# Autodesk Inventor assembly: Assembly1
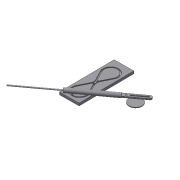
[picture p0: Inventor's stored thumbnail of the model, 180x180]
Saved by Autodesk Inventor 2017 (Build 210142000, 142)
## iProperties
Created: 2019-07-04
Part Number: Assembly1
Document SubType Name: Assembly
Designer: Admin
Author: Admin
## Documents named in this file (7)
- E:\PK\8 mechanism\Prototype 2\Assembly1.iam
- E:\PK\8 mechanism\Prototype 2\Part1.ipt
- E:\PK\8 mechanism\Prototype 2\Part2.ipt
- E:\PK\8 mechanism\Prototype 2\Part3.ipt
- E:\PK\8 mechanism\Prototype 2\Part4.ipt
- E:\PK\8 mechanism\Prototype 2\Part5.ipt
- E:\PK\8 mechanism\Prototype 2\Part12.ipt
## Components (8 placed, 6 different names)
1. Part1:1 — Mate:1, Flush:1, Flush:2, Tangent:1, Mate:3, Angle:1, Mate:5
2. Part2:1 — Mate:1, Flush:1
3. Part2:2 — Flush:2, Mate:4
4. Part3:1 — Tangent:1, Mate:2, Tangent:2, Mate:4, Angle:1, Mate:5
5. Part4:1 — Mate:2, Tangent:2, Transitional:1
6. Part5:1 — Mate:3, Insert:2, Insert:3, Transitional:1, Rotational:1, Rotational:2
7. Part12:1 — Insert:3, Rotational:1
8. Part12:2 — Insert:2, Rotational:2
## Relationships (15: Mate 5, Flush 2, Tangent 2, Insert 2, RevoluteJoint 2, Angle 1, Transitional 1)
- Mate:1: Part1:1 ↔ Part2:1
- Flush:1 (-10 mm): Part1:1 ↔ Part2:1
- Flush:2: Part1:1 ↔ Part2:2
- Tangent:1: Part1:1 ↔ Part3:1
- Mate:2: Part3:1 ↔ Part4:1
- Tangent:2: Part3:1 ↔ Part4:1
- Mate:3 (20 mm): Part1:1 ↔ Part5:1
- Insert:2: Part5:1 ↔ Part12:2
- Insert:3: Part5:1 ↔ Part12:1
- Mate:4: Part2:2 ↔ Part3:1
- Angle:1 (180 deg): Part1:1 ↔ Part3:1
- Mate:5: Part1:1 ↔ Part3:1
- Transitional:1: Part4:1 ↔ Part5:1
- Rotational:1 [RevoluteJoint]: Part5:1 ↔ Part12:1
- Rotational:2 [RevoluteJoint]: Part5:1 ↔ Part12:2
